# Autodesk Inventor assembly: Mold Design1
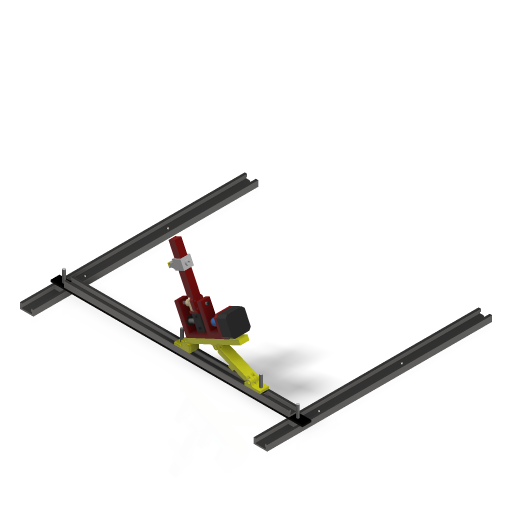
[picture p0: Inventor's stored thumbnail of the model, 512x512]
Saved by Autodesk Inventor 2024 (Build 280153000, 153)
## iProperties
Created: 2023-04-17
Part Number: Mold Design1
Document SubType Name: Assembly
Designer: ferna
Author: ferna
## Documents named in this file (8)
- C:\Users\ferna\OneDrive - Universidad Católica de Chile\Bocas\RobotFlautista\Mold Design1\Mold Design1.iam
- C:\Users\ferna\OneDrive - Universidad Católica de Chile\Bocas\NuevosDedos\Dedo - 1.iam
- C:\Users\ferna\OneDrive - Universidad Católica de Chile\Bocas\NuevosDedos\Lifter 1.iam
- C:\Users\ferna\OneDrive - Universidad Católica de Chile\Bocas\NuevosDedos\MedioRielT-Track.ipt
- C:\Users\ferna\OneDrive - Universidad Católica de Chile\Bocas\NuevosDedos\PaloBase.ipt
- C:\Users\ferna\OneDrive - Universidad Católica de Chile\Bocas\NuevosDedos\AprietaRielT.ipt
- C:\Users\ferna\OneDrive - Universidad Católica de Chile\Bocas\NuevosDedos\CuarentaRielT-Track.ipt
- C:\Users\ferna\OneDrive - Universidad Católica de Chile\Bocas\NuevosDedos\AprietaRielTChico.ipt
## Components (10 placed, 7 different names)
1. Dedo - 1:1 [sub-assembly] — Mate:1, Flush:1, Flush:2
2. Lifter 1:1 [sub-assembly] — Mate:1, Flush:1, Flush:2, Mate:10, Mate:11, Mate:14
3. MedioRielT-Track:1
4. MedioRielT-Track:2
5. PaloBase:1
6. AprietaRielT:1
7. AprietaRielT:2
8. CuarentaRielT-Track:1 — Mate:12, Mate:13, Angle:3, Angle:4, Mate:15, Mate:16
9. AprietaRielTChico:1 — Mate:10, Mate:13, Angle:4, Mate:15
10. AprietaRielTChico:2 — Mate:11, Mate:12, Angle:3, Mate:14, Mate:16
## Relationships (25: Mate 16, Flush 5, Angle 4)
- Mate:1: Dedo - 1:1 ↔ Lifter 1:1
- Flush:1: Dedo - 1:1 ↔ Lifter 1:1
- Flush:2: Dedo - 1:1 ↔ Lifter 1:1
- [Mate] (0.3 mm): MedioRielT-Track:1 ↔ AprietaRielT:1
- [Mate] (0.3 mm): MedioRielT-Track:1 ↔ AprietaRielT:1
- [Mate]: PaloBase:1 ↔ AprietaRielT:1
- [Mate]: MedioRielT-Track:1 ↔ PaloBase:1
- [Angle] (0 deg): MedioRielT-Track:1 ↔ PaloBase:1
- [Mate]: PaloBase:1 ↔ AprietaRielT:2
- [Mate]: MedioRielT-Track:2 ↔ AprietaRielT:2
- [Flush]: MedioRielT-Track:1 ↔ MedioRielT-Track:2
- [Mate] (0.3 mm): MedioRielT-Track:2 ↔ AprietaRielT:2
- [Angle] (0 deg): MedioRielT-Track:2 ↔ PaloBase:1
- [Mate]: PaloBase:1 ↔ CuarentaRielT-Track:1
- [Flush]: PaloBase:1 ↔ CuarentaRielT-Track:1
- [Flush] (30 mm): PaloBase:1 ↔ CuarentaRielT-Track:1
- Mate:10: Lifter 1:1 ↔ AprietaRielTChico:1
- Mate:11: Lifter 1:1 ↔ AprietaRielTChico:2
- Mate:12: CuarentaRielT-Track:1 ↔ AprietaRielTChico:2
- Mate:13: CuarentaRielT-Track:1 ↔ AprietaRielTChico:1
- Angle:3 (0 deg): CuarentaRielT-Track:1 ↔ AprietaRielTChico:2
- Angle:4 (0 deg): CuarentaRielT-Track:1 ↔ AprietaRielTChico:1
- Mate:14: Lifter 1:1 ↔ AprietaRielTChico:2
- Mate:15 (0.125 mm): CuarentaRielT-Track:1 ↔ AprietaRielTChico:1
- Mate:16 (0.125 mm): CuarentaRielT-Track:1 ↔ AprietaRielTChico:2
## Named parameters: d3_d4 = 0.3 mm, d4_d5 = 0.3 mm, d5_d6 = 0 mm, d6_d7 = 0 mm, d7_d8 = 0 deg, d8_d9 = 0 mm, d9_d10 = 0 mm, d10_d12 = 0 mm, d11_d13 = 0.3 mm, d12_d14 = 0 deg, d13_d15 = 0 mm
